# Autodesk Inventor assembly: MTLV-S03
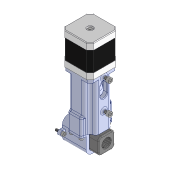
[picture p0: Inventor's stored thumbnail of the model, 180x180]
Saved by Autodesk Inventor 2020 (Build 240168000, 168)
## iProperties
Created: 2020-03-28
Part Number: MTLV-S03
Document SubType Name: Assembly
Designer: John K
Author: John K
## Documents named in this file (8)
- C:\GrabCAD\MTL Ventilator Design\MTLV\Subassemblies\MTLV-S03.iam
- C:\GrabCAD\MTL Ventilator Design\MTLV\Commercial Parts\Flow-Related\Needle Valve 4891K72.ipt
- C:\GrabCAD\MTL Ventilator Design\MTLV\Manufactured Parts\MTLV-P15.ipt
- C:\GrabCAD\MTL Ventilator Design\MTLV\Manufactured Parts\MTLV-P16.ipt
- C:\GrabCAD\MTL Ventilator Design\MTLV\Manufactured Parts\MTLV-P17.ipt
- C:\GrabCAD\MTL Ventilator Design\MTLV\Commercial Parts\Electronics\Stepper Motor NEMA17 v40.ipt
- C:\GrabCAD\MTL Ventilator Design\MTLV\Commercial Parts\Fasteners\M3x10mm Socket.ipt
- C:\GrabCAD\MTL Ventilator Design\MTLV\Commercial Parts\Fasteners\M4x12mm Socket.ipt
## Components (14 placed, 7 different names)
1. Needle Valve 4891K72:1 — Mate:1, Mate:2, Mate:3, Mate:4, Mate:5, Mate:6
2. MTLV-P15:1 — Mate:1, Mate:2, Mate:7, Mate:8, Insert:1, Insert:2, Insert:3, Insert:6, Insert:7, Insert:8, Insert:9
3. MTLV-P16:1 — Mate:3, Mate:4, Mate:5, Mate:9
4. MTLV-P17:1 — Mate:6, Mate:7, Mate:8, Mate:10, Mate:11, Insert:4, Insert:5
5. Stepper Motor NEMA17 v40:1 — Mate:9, Mate:10, Mate:11
6. M4x12mm Socket:1 — Insert:4
7. M4x12mm Socket:2 — Insert:5
8. M3x10mm Socket:4 — Insert:6
9. M3x10mm Socket:5 — Insert:7
10. M3x10mm Socket:6 — Insert:8
11. M3x10mm Socket:7 — Insert:9
12. M3x10mm Socket:1 — Insert:1
13. M3x10mm Socket:2 — Insert:2
14. M3x10mm Socket:3 — Insert:3
## Relationships (20: Mate 11, Insert 9)
- Mate:1: Needle Valve 4891K72:1 ↔ MTLV-P15:1
- Mate:2: Needle Valve 4891K72:1 ↔ MTLV-P15:1
- Mate:3: Needle Valve 4891K72:1 ↔ MTLV-P16:1
- Mate:4: Needle Valve 4891K72:1 ↔ MTLV-P16:1
- Mate:5: Needle Valve 4891K72:1 ↔ MTLV-P16:1
- Mate:6: Needle Valve 4891K72:1 ↔ MTLV-P17:1
- Mate:7: MTLV-P15:1 ↔ MTLV-P17:1
- Mate:8: MTLV-P15:1 ↔ MTLV-P17:1
- Mate:9: MTLV-P16:1 ↔ Stepper Motor NEMA17 v40:1
- Mate:10: MTLV-P17:1 ↔ Stepper Motor NEMA17 v40:1
- Mate:11: MTLV-P17:1 ↔ Stepper Motor NEMA17 v40:1
- Insert:1: MTLV-P15:1 ↔ M3x10mm Socket:1
- Insert:2: MTLV-P15:1 ↔ M3x10mm Socket:2
- Insert:3: MTLV-P15:1 ↔ M3x10mm Socket:3
- Insert:4 (4.1 mm): MTLV-P17:1 ↔ M4x12mm Socket:1
- Insert:5 (4.1 mm): MTLV-P17:1 ↔ M4x12mm Socket:2
- Insert:6: MTLV-P15:1 ↔ M3x10mm Socket:4
- Insert:7: MTLV-P15:1 ↔ M3x10mm Socket:5
- Insert:8: MTLV-P15:1 ↔ M3x10mm Socket:6
- Insert:9: MTLV-P15:1 ↔ M3x10mm Socket:7
